# Autodesk Inventor assembly: final 3
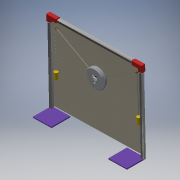
[picture p0: Inventor's stored thumbnail of the model, 180x180]
Saved by Autodesk Inventor 2019 (Build 230136000, 136)
## iProperties
Created: 2020-02-12
Part Number: final 3
Document SubType Name: Assembly
Designer: Vinayak
Author: Vinayak
## Documents named in this file (12)
- C:\Users\Vinayak\Documents\3d inventor\final 3.iam
- C:\Users\Vinayak\Documents\3d inventor\elbow.ipt
- C:\Users\Vinayak\Documents\3d inventor\frame.ipt
- C:\Users\Vinayak\Documents\3d inventor\foot.ipt
- C:\Users\Vinayak\Documents\3d inventor\left motor pulley.iam
- C:\Users\Vinayak\Documents\3d inventor\right motor pulley.iam
- C:\Users\Vinayak\Documents\3d inventor\belt new.ipt
- C:\Users\Vinayak\Documents\3d inventor\Part1.ipt
- C:\Users\Vinayak\Documents\3d inventor\gond.ipt
- C:\Users\Vinayak\Documents\3d inventor\wiegth and belt.iam
- C:\Users\Vinayak\Documents\serfvo motor.iam
- C:\Users\Vinayak\Documents\sheet.ipt
## Components (27 placed, 11 different names)
1. elbow:1 — Rigid:1, Rigid:4, Rigid:28
2. elbow:2 — Rigid:2, Rigid:3, Rigid:27, Rigid:29
3. frame:1 — Rigid:4, Rigid:5
4. frame:2 — Rigid:1, Rigid:2, Rigid:27, Rigid:45
5. frame:3 — Rigid:3, Rigid:6
6. foot:1 — Rigid:5
7. foot:2 — Rigid:6
8. Part1:1
9. right motor pulley:1 [sub-assembly] — Rigid:28, Rigid:30, Rigid:40
10. left motor pulley:1 [sub-assembly] — Rigid:29, Rigid:34, Rigid:38
11. belt new:1 — Rigid:30, Rigid:31
12. belt new:4 — Rigid:41, Rigid:42
13. belt new:5 — Rigid:31, Rigid:32
14. belt new:6 — Rigid:32, Rigid:33
15. belt new:7 — Rigid:33
16. belt new:8 — Rigid:36, Rigid:37
17. belt new:9 — Rigid:34, Rigid:35
18. belt new:10 — Rigid:38, Rigid:39
19. belt new:11 — Rigid:40, Rigid:41
20. belt new:12 — Rigid:39, Rigid:43
21. belt new:13 — Rigid:35, Rigid:36
22. belt new:14 — Rigid:37, Mate:1
23. gond:1 — Mate:1, Rigid:44
24. wiegth and belt:1 [sub-assembly] — Rigid:42
25. wiegth and belt:2 [sub-assembly] — Rigid:43
26. serfvo motor:1 [sub-assembly] — Rigid:44
27. sheet:1 — Rigid:45
## Relationships (26: WeldJoint 25, Mate 1)
- Rigid:1 [WeldJoint]: elbow:1 ↔ frame:2
- Rigid:2 [WeldJoint]: elbow:2 ↔ frame:2
- Rigid:3 [WeldJoint]: elbow:2 ↔ frame:3
- Rigid:4 [WeldJoint]: elbow:1 ↔ frame:1
- Rigid:5 [WeldJoint]: frame:1 ↔ foot:1
- Rigid:6 [WeldJoint]: frame:3 ↔ foot:2
- Rigid:27 [WeldJoint]: elbow:2 ↔ frame:2
- Rigid:28 [WeldJoint]: elbow:1 ↔ right motor pulley:1
- Rigid:29 [WeldJoint]: elbow:2 ↔ left motor pulley:1
- Rigid:30 [WeldJoint]: right motor pulley:1 ↔ belt new:1
- Rigid:31 [WeldJoint]: belt new:1 ↔ belt new:5
- Rigid:32 [WeldJoint]: belt new:5 ↔ belt new:6
- Rigid:33 [WeldJoint]: belt new:6 ↔ belt new:7
- Rigid:34 [WeldJoint]: left motor pulley:1 ↔ belt new:9
- Rigid:35 [WeldJoint]: belt new:9 ↔ belt new:13
- Rigid:36 [WeldJoint]: belt new:8 ↔ belt new:13
- Rigid:37 [WeldJoint]: belt new:8 ↔ belt new:14
- Mate:1: belt new:14 ↔ gond:1
- Rigid:38 [WeldJoint]: left motor pulley:1 ↔ belt new:10
- Rigid:39 [WeldJoint]: belt new:10 ↔ belt new:12
- Rigid:40 [WeldJoint]: right motor pulley:1 ↔ belt new:11
- Rigid:41 [WeldJoint]: belt new:4 ↔ belt new:11
- Rigid:42 [WeldJoint]: belt new:4 ↔ wiegth and belt:1
- Rigid:43 [WeldJoint]: belt new:12 ↔ wiegth and belt:2
- Rigid:44 [WeldJoint]: gond:1 ↔ serfvo motor:1
- Rigid:45 [WeldJoint]: frame:2 ↔ sheet:1
